# Autodesk Inventor assembly: DcMotor
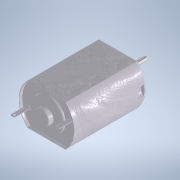
[picture p0: Inventor's stored thumbnail of the model, 180x180]
Saved by Autodesk Inventor 2021 (Build 250183000, 183)
## iProperties
Created: 2022-02-21
Part Number: DcMotor
Document SubType Name: Assembly
Designer: 12491
Author: 12491
## Documents named in this file (3)
- C:\Users\12491\Desktop\StructProject\DCFanShelf\DcMotor.iam
- C:\Users\12491\Desktop\StructProject\DCFanShelf\DcMotor_Body.ipt
- C:\Users\12491\Desktop\StructProject\DCFanShelf\DcMotor_Shift.ipt
## Components (2 placed, 2 different names)
1. DcMotor_Body:1 — 表面齐平:1, 表面齐平:2, 表面齐平:3, 配合:1, 插入:1
2. DcMotor_Shift:1 — 配合:1, 插入:1
## Relationships (5: Flush 3, Mate 1, Insert 1)
- 表面齐平:1 [Flush]: DcMotor_Body:1
- 表面齐平:2 [Flush]: DcMotor_Body:1
- 表面齐平:3 [Flush]: DcMotor_Body:1
- 配合:1 [Mate]: DcMotor_Body:1 ↔ DcMotor_Shift:1
- 插入:1 [Insert]: DcMotor_Body:1 ↔ DcMotor_Shift:1
